# Autodesk Inventor assembly: Box2
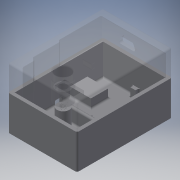
[picture p0: Inventor's stored thumbnail of the model, 180x180]
Saved by Autodesk Inventor 2019 (Build 230136000, 136)
## iProperties
Created: 2020-09-23
Part Number: Box2
Document SubType Name: Assembly
Designer: Vincent
Author: Vincent
## Documents named in this file (3)
- C:\Vincent\Postdoc\Melbourne\Fourier\The University of Melbourne\Justin Fong - FourierJointLab\ShoulderTrackingStudy\Tech\Hardware\Box2.iam
- C:\Vincent\Postdoc\Melbourne\Fourier\The University of Melbourne\Justin Fong - FourierJointLab\ShoulderTrackingStudy\Tech\Hardware\BoxLid2.ipt
- C:\Vincent\Postdoc\Melbourne\Fourier\The University of Melbourne\Justin Fong - FourierJointLab\ShoulderTrackingStudy\Tech\Hardware\BoxBottom2.ipt
## Components (2 placed, 2 different names)
1. BoxLid2:1 — Mate:1, Mate:2, Mate:3
2. BoxBottom2:1 — Mate:1, Mate:2, Mate:3
## Relationships (3: Mate 3)
- Mate:1: BoxLid2:1 ↔ BoxBottom2:1
- Mate:2: BoxLid2:1 ↔ BoxBottom2:1
- Mate:3: BoxLid2:1 ↔ BoxBottom2:1
